# Autodesk Inventor assembly: КВ33.044.300 -  Сборка мотора Makeblock с крепление
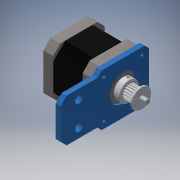
[picture p0: Inventor's stored thumbnail of the model, 180x180]
Saved by Autodesk Inventor 2019 (Build 230136000, 136)
## iProperties
Created: 2019-07-17
Part Number: КВ33.044.300 -  Сборка мотора Makeblock с крепление
Material: Типовые
Document SubType Name: Assembly
Designer: Петров Иван
Author: Петров Иван
## Documents named in this file (4)
- E:\IVAN\Kvantoriada2019\optimal_gripper\hardware\КВ33.044.300 -  Сборка мотора Makeblock с крепление.iam
- E:\IVAN\Kvantoriada2019\optimal_gripper\hardware\КВ33.044.301 - Деражатель мотора.ipt
- E:\IVAN\Kvantoriada2019\optimal_gripper\hardware\Стандартные изделия\Шаговый двигатель Makeblock.ipt
- E:\IVAN\Kvantoriada2019\optimal_gripper\hardware\Стандартные изделия\шкив Makeblock.ipt
## Components (3 placed, 3 different names)
1. КВ33.044.301 - Деражатель мотора:1 — Совмещение:1, Совмещение:2, Совмещение:3, Совмещение:5
2. Шаговый двигатель Makeblock:1 — Совмещение:1, Совмещение:2, Совмещение:3, Совмещение:4
3. шкив Makeblock:1 — Совмещение:4, Совмещение:5
## Relationships (5: Mate 5)
- Совмещение:1 [Mate]: КВ33.044.301 - Деражатель мотора:1 ↔ Шаговый двигатель Makeblock:1
- Совмещение:2 [Mate]: КВ33.044.301 - Деражатель мотора:1 ↔ Шаговый двигатель Makeblock:1
- Совмещение:3 [Mate]: КВ33.044.301 - Деражатель мотора:1 ↔ Шаговый двигатель Makeblock:1
- Совмещение:4 [Mate]: Шаговый двигатель Makeblock:1 ↔ шкив Makeblock:1
- Совмещение:5 [Mate]: КВ33.044.301 - Деражатель мотора:1 ↔ шкив Makeblock:1
